# Autodesk Inventor assembly: body assy
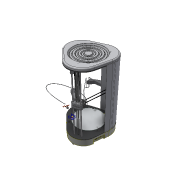
[picture p0: Inventor's stored thumbnail of the model, 180x180]
Saved by Autodesk Inventor 2016 (Build 200138000, 138)
## iProperties
Created: 2016-12-29
Part Number: body assy
Document SubType Name: Assembly
Designer: admin
Author: admin
## Documents named in this file (32)
- C:\Users\Juny\Desktop\Ateam\1612 3D 도면\body assy VER2.iam
- C:\Users\Juny\Desktop\Ateam\1612 3D 도면\head_cable_holder.ipt
- C:\Users\Juny\Desktop\Ateam\1612 3D 도면\m3 6 socket_screw.ipt
- C:\Users\Juny\Desktop\Ateam\1612 3D 도면\m3 8 socket_screw.ipt
- C:\Users\Juny\Desktop\Ateam\1612 3D 도면\M3 16 BH_tapping_screw.ipt
- C:\Users\Juny\Desktop\Ateam\1612 3D 도면\m3 30 pcb_support.ipt
- C:\Users\Juny\Desktop\Ateam\1612 3D 도면\m4 10 Button Head.ipt
- C:\Users\Juny\Desktop\Ateam\1612 3D 도면\m4 12 Button Head.ipt
- C:\Users\Juny\Desktop\Ateam\1612 3D 도면\m4 20 Button Head.ipt
- C:\Users\Juny\Desktop\Ateam\1612 3D 도면\main_board.ipt
- C:\Users\Juny\Desktop\Ateam\1612 3D 도면\post.ipt
- C:\Users\Juny\Desktop\Ateam\1612 3D 도면\timing_belt.ipt
- C:\Users\Juny\Desktop\Ateam\1612 3D 도면\top_cover.ipt
- C:\Users\Juny\Desktop\Ateam\1612 3D 도면\back_cover.ipt
- C:\Users\Juny\Desktop\Ateam\1612 3D 도면\bottom cover assy\bottom cover assy.iam
- C:\Users\Juny\Desktop\Ateam\1612 3D 도면\bottom plate assy\bottom plate assy.iam
- C:\Users\Juny\Desktop\Ateam\1612 3D 도면\head assy\head assy.iam
- C:\Users\Juny\Desktop\Ateam\1612 3D 도면\lift block assy\lift block assy.iam
- C:\Users\Juny\Desktop\Ateam\1612 3D 도면\lod assy\lod assy.iam
- C:\Users\Juny\Desktop\Ateam\1612 3D 도면\motor assy\motor assy.iam
- C:\Users\Juny\Desktop\Ateam\1612 3D 도면\oled assy\oled assy.iam
- C:\Users\Juny\Desktop\Ateam\1612 3D 도면\top plate assy\top plate assy.iam
- C:\Users\Juny\Desktop\Ateam\1612 3D 도면\-another-(개발시 참고)\hanger.ipt
- C:\Users\Juny\Desktop\Ateam\1612 3D 도면\-another-(개발시 참고)\cusion.ipt
- C:\Users\Juny\Desktop\Ateam\1612 3D 도면\head assy\nozzle0.6.ipt
- C:\Users\Juny\Desktop\Ateam\1612 3D 도면\head assy\nozzle0.8.ipt
- C:\Users\Juny\Desktop\Ateam\1612 3D 도면\head assy\nozzle0.25.ipt
- C:\Users\Juny\Desktop\Ateam\1612 3D 도면\-another-(개발시 참고)\tube.ipt
- C:\Users\Juny\Desktop\Ateam\1612 3D 도면\bottom cover assy\bottom_cover VER.2 LCD.ipt
- C:\Users\Juny\Desktop\Ateam\1612 3D 도면\bottom cover assy\VER.2 LCD.ipt
- C:\Users\Juny\Desktop\Ateam\1612 3D 도면\bottom cover assy\filter ver1.ipt
- C:\Users\Juny\Desktop\Ateam\1612 3D 도면\bottom cover assy\8025 fan.ipt
## Components (76 placed, 31 different names)
1. head_cable_holder:1
2. m3 6 socket_screw:1 — Rotational:39
3. M3 16 BH_tapping_screw:1 — Rotational:18
4. m3 30 pcb_support:1 — Rotational:33
5. m4 10 Button Head:1 — Rotational:25
6. m4 12 Button Head:1 — Rotational:32
7. main_board:1 — Rotational:37, Rotational:38, Rotational:39, Rotational:40, Rotational:41, Rotational:42
8. top_cover:1 — Rotational:23, Rotational:24
9. back_cover:1 — Rotational:21, Rotational:22, Rotational:25, Rotational:26, Rotational:27, Rotational:28, Rotational:29, Rotational:30, Rotational:31, Rotational:32
10. bottom cover assy:1 [sub-assembly] — Rotational:43, Rotational:44
11. bottom plate assy:1 [sub-assembly] — Rotational:3, Rotational:4, Rotational:5, Rotational:6, Rotational:7, Rotational:8, Rotational:21, Rotational:22, Angle:1, Angle:3, Angle:4, Rotational:33, Rotational:34, Rotational:35, Rotational:36, Rotational:43, Rotational:44, Mate:4, Mate:6
12. head assy:1 [sub-assembly] — Tangent:7, Tangent:8, Tangent:9, Tangent:10, Tangent:11, Tangent:12
13. lod assy:1 [sub-assembly] — Tangent:1, Tangent:8
14. oled assy:1 [sub-assembly] — Rotational:5, Rotational:6, Rotational:14, Rotational:15, Rotational:16, Rotational:17
15. top plate assy:1 [sub-assembly] — Rotational:1, Rotational:2, Rotational:11, Rotational:12, Rotational:13, Rotational:18, Rotational:19, Rotational:20, Rotational:23, Rotational:24
16. m3 8 socket_screw:2 — Rotational:14
17. m3 8 socket_screw:3 — Rotational:15
18. m3 8 socket_screw:4 — Rotational:16
19. m3 8 socket_screw:5 — Rotational:17
20. M3 16 BH_tapping_screw:2 — Rotational:19
21. M3 16 BH_tapping_screw:3 — Rotational:20
22. lift block assy:1 [sub-assembly] — Mate:1, Angle:1, Tangent:1, Tangent:2
23. lift block assy:2 [sub-assembly] — Mate:3, Angle:4, Tangent:3, Tangent:4
24. lift block assy:3 [sub-assembly] — Mate:2, Angle:3, Tangent:5, Tangent:6
25. m4 10 Button Head:2 — Rotational:26
26. m4 10 Button Head:3 — Rotational:27
27. m4 10 Button Head:4 — Rotational:28
28. m4 12 Button Head:2 — Rotational:31
29. m4 12 Button Head:3 — Rotational:30
30. m4 12 Button Head:4 — Rotational:29
31. m3 30 pcb_support:2 — Rotational:36
32. m3 30 pcb_support:3 — Rotational:35, Rotational:37
33. m3 30 pcb_support:4 — Rotational:34, Rotational:38
34. m3 6 socket_screw:2 — Rotational:40
35. m3 6 socket_screw:3 — Rotational:41
36. m3 6 socket_screw:4 — Rotational:42
37. lod assy:2 [sub-assembly] — Tangent:2, Tangent:7
38. lod assy:3 [sub-assembly] — Tangent:3, Tangent:11
39. lod assy:4 [sub-assembly] — Tangent:4, Tangent:12
40. lod assy:5 [sub-assembly] — Tangent:5, Tangent:10
41. lod assy:6 [sub-assembly] — Tangent:6, Tangent:9
42. head_cable_holder:2
43. hanger:1
44. cusion:1
45. nozzle0.6:1
46. nozzle0.8:1
47. nozzle0.25:1
48. tube:1
49. bottom_cover VER.2 LCD:1 — Mate:4, Mate:5, Mate:6
50. VER.2 LCD:1 — Mate:5
51. filter ver1:1
52. 8025 fan:1
53. post:2 — Rotational:1, Rotational:3, Mate:2
54. timing_belt:1 — Rotational:13, Cylindrical:1
55. post:1 — Rotational:2, Rotational:4
56. m4 20 Button Head:4 — Rotational:12
57. m4 20 Button Head:3 — Rotational:11
58. m4 20 Button Head:1 — Rotational:9
59. m4 20 Button Head:2 — Rotational:10
60. motor assy:1 [sub-assembly] — Rotational:7, Rotational:8, Rotational:9, Rotational:10, Cylindrical:1
61. post:3 — Mate:3
62. timing_belt:2
63. post:4
64. m4 20 Button Head:5
65. m4 20 Button Head:6
66. m4 20 Button Head:7
67. m4 20 Button Head:8
68. motor assy:2 [sub-assembly]
69. post:5
70. timing_belt:3
71. post:6 — Mate:1
72. m4 20 Button Head:9
73. m4 20 Button Head:10
74. m4 20 Button Head:11
75. m4 20 Button Head:12
76. motor assy:3 [sub-assembly]
## Component patterns: (3 elements, first: post:2 + timing_belt:1 + post:1 + m4 20 Button Head:4 + m4 20 Button Head:3 + m4 20 Button Head:1 + m4 20 Button Head:2 + motor assy:1)
## Relationships (66: RevoluteJoint 44, Tangent 12, Mate 6, Angle 3, CylindricalJoint 1)
- Rotational:1 [RevoluteJoint]: top plate assy:1 ↔ post:2
- Rotational:2 [RevoluteJoint]: top plate assy:1 ↔ post:1
- Rotational:3 [RevoluteJoint]: bottom plate assy:1 ↔ post:2
- Rotational:4 [RevoluteJoint]: bottom plate assy:1 ↔ post:1
- Rotational:5 [RevoluteJoint]: bottom plate assy:1 ↔ oled assy:1
- Rotational:6 [RevoluteJoint]: bottom plate assy:1 ↔ oled assy:1
- Rotational:7 [RevoluteJoint]: bottom plate assy:1 ↔ motor assy:1
- Rotational:8 [RevoluteJoint]: bottom plate assy:1 ↔ motor assy:1
- Rotational:9 [RevoluteJoint]: m4 20 Button Head:1 ↔ motor assy:1
- Rotational:10 [RevoluteJoint]: m4 20 Button Head:2 ↔ motor assy:1
- Rotational:11 [RevoluteJoint]: top plate assy:1 ↔ m4 20 Button Head:3
- Rotational:12 [RevoluteJoint]: top plate assy:1 ↔ m4 20 Button Head:4
- Rotational:13 [RevoluteJoint]: top plate assy:1 ↔ timing_belt:1
- Cylindrical:1: timing_belt:1 ↔ motor assy:1
- Rotational:14 [RevoluteJoint]: oled assy:1 ↔ m3 8 socket_screw:2
- Rotational:15 [RevoluteJoint]: oled assy:1 ↔ m3 8 socket_screw:3
- Rotational:16 [RevoluteJoint]: oled assy:1 ↔ m3 8 socket_screw:4
- Rotational:17 [RevoluteJoint]: oled assy:1 ↔ m3 8 socket_screw:5
- Rotational:18 [RevoluteJoint]: M3 16 BH_tapping_screw:1 ↔ top plate assy:1
- Rotational:19 [RevoluteJoint]: top plate assy:1 ↔ M3 16 BH_tapping_screw:2
- Rotational:20 [RevoluteJoint]: top plate assy:1 ↔ M3 16 BH_tapping_screw:3
- Rotational:21 [RevoluteJoint]: back_cover:1 ↔ bottom plate assy:1
- Rotational:22 [RevoluteJoint]: back_cover:1 ↔ bottom plate assy:1
- Rotational:23 [RevoluteJoint]: top_cover:1 ↔ top plate assy:1
- Rotational:24 [RevoluteJoint]: top_cover:1 ↔ top plate assy:1
- Mate:1: lift block assy:1 ↔ post:6
- Angle:1 (0 deg): bottom plate assy:1 ↔ lift block assy:1
- Mate:2: lift block assy:3 ↔ post:2
- Angle:3 (0 deg): bottom plate assy:1 ↔ lift block assy:3
- Mate:3: lift block assy:2 ↔ post:3
- Angle:4 (0 deg): bottom plate assy:1 ↔ lift block assy:2
- Rotational:25 [RevoluteJoint]: m4 10 Button Head:1 ↔ back_cover:1
- Rotational:26 [RevoluteJoint]: back_cover:1 ↔ m4 10 Button Head:2
- Rotational:27 [RevoluteJoint]: back_cover:1 ↔ m4 10 Button Head:3
- Rotational:28 [RevoluteJoint]: back_cover:1 ↔ m4 10 Button Head:4
- Rotational:29 [RevoluteJoint]: back_cover:1 ↔ m4 12 Button Head:4
- Rotational:30 [RevoluteJoint]: back_cover:1 ↔ m4 12 Button Head:3
- Rotational:31 [RevoluteJoint]: back_cover:1 ↔ m4 12 Button Head:2
- Rotational:32 [RevoluteJoint]: m4 12 Button Head:1 ↔ back_cover:1
- Rotational:33 [RevoluteJoint]: m3 30 pcb_support:1 ↔ bottom plate assy:1
- Rotational:34 [RevoluteJoint]: bottom plate assy:1 ↔ m3 30 pcb_support:4
- Rotational:35 [RevoluteJoint]: bottom plate assy:1 ↔ m3 30 pcb_support:3
- Rotational:36 [RevoluteJoint]: bottom plate assy:1 ↔ m3 30 pcb_support:2
- Rotational:37 [RevoluteJoint]: main_board:1 ↔ m3 30 pcb_support:3
- Rotational:38 [RevoluteJoint]: main_board:1 ↔ m3 30 pcb_support:4
- Rotational:39 [RevoluteJoint]: m3 6 socket_screw:1 ↔ main_board:1
- Rotational:40 [RevoluteJoint]: main_board:1 ↔ m3 6 socket_screw:2
- Rotational:41 [RevoluteJoint]: main_board:1 ↔ m3 6 socket_screw:3
- Rotational:42 [RevoluteJoint]: main_board:1 ↔ m3 6 socket_screw:4
- Rotational:43 [RevoluteJoint]: bottom cover assy:1 ↔ bottom plate assy:1
- Rotational:44 [RevoluteJoint]: bottom cover assy:1 ↔ bottom plate assy:1
- Tangent:1: lod assy:1 ↔ lift block assy:1
- Tangent:2: lift block assy:1 ↔ lod assy:2
- Tangent:3: lift block assy:2 ↔ lod assy:3
- Tangent:4: lift block assy:2 ↔ lod assy:4
- Tangent:5: lift block assy:3 ↔ lod assy:5
- Tangent:6: lift block assy:3 ↔ lod assy:6
- Tangent:7: head assy:1 ↔ lod assy:2
- Tangent:8: head assy:1 ↔ lod assy:1
- Tangent:9: head assy:1 ↔ lod assy:6
- Tangent:10: head assy:1 ↔ lod assy:5
- Tangent:11: head assy:1 ↔ lod assy:3
- Tangent:12: head assy:1 ↔ lod assy:4
- Mate:4: bottom plate assy:1 ↔ bottom_cover VER.2 LCD:1
- Mate:5: bottom_cover VER.2 LCD:1 ↔ VER.2 LCD:1
- Mate:6: bottom plate assy:1 ↔ bottom_cover VER.2 LCD:1
